# Autodesk Inventor assembly: компановка новая
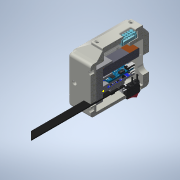
[picture p0: Inventor's stored thumbnail of the model, 180x180]
Saved by Autodesk Inventor 2021 (Build 250183000, 183)
## iProperties
Created: 2023-02-11
Part Number: компановка новая
Document SubType Name: Assembly
Designer: Tasya
Mass: 94.4631 g
Surface Area: 527.261 cm^2
Volume: 88.6889 cm^3
Density: 1.06511 g/cm^3
Author: Tasya
## Documents named in this file (6)
- C:\Users\Tasya\Desktop\теплица\3D модели\компановка новая.iam
- C:\Users\Tasya\Desktop\теплица\датчики почва воздух\корпус.ipt
- C:\Users\Tasya\Desktop\теплица\датчики почва воздух\DHT11.ipt
- C:\Users\Tasya\Desktop\теплица\датчики почва воздух\крышка корпус.ipt
- C:\Users\Tasya\Desktop\теплица\grabcad\Switch on off.ipt
- C:\Users\Tasya\Desktop\теплица\датчики почва воздух\Компоновка.iam
## Components (5 placed, 5 different names)
1. корпус:1 — Совмещение:1, Совмещение:2, Совмещение:3, Совмещение:4, Совмещение:8, Совмещение:9, Совмещение:11, Совмещение:12, Совмещение:13, Совмещение:14, Совмещение:15
2. DHT11:1 — Совмещение:1, Совмещение:2, Совмещение:3
3. крышка корпус:1 — Совмещение:4, Совмещение:8, Совмещение:9
4. Switch on off:1 — Совмещение:11, Совмещение:12, Совмещение:13
5. Компоновка:1 [sub-assembly] — Совмещение:10, Угол:1, Совмещение:14, Совмещение:15
## Relationships (13: Mate 12, Angle 1)
- Совмещение:1 [Mate] (1 mm): корпус:1 ↔ DHT11:1
- Совмещение:2 [Mate] (1 mm): корпус:1 ↔ DHT11:1
- Совмещение:3 [Mate] (0.5 mm): корпус:1 ↔ DHT11:1
- Совмещение:4 [Mate]: корпус:1 ↔ крышка корпус:1
- Совмещение:8 [Mate]: корпус:1 ↔ крышка корпус:1
- Совмещение:9 [Mate]: корпус:1 ↔ крышка корпус:1
- Совмещение:10 [Mate]: Компоновка:1
- Угол:1 [Angle] (180 deg): Компоновка:1
- Совмещение:11 [Mate]: корпус:1 ↔ Switch on off:1
- Совмещение:12 [Mate] (1.7 mm): корпус:1 ↔ Switch on off:1
- Совмещение:13 [Mate]: корпус:1 ↔ Switch on off:1
- Совмещение:14 [Mate]: корпус:1 ↔ Компоновка:1
- Совмещение:15 [Mate] (1 mm): корпус:1 ↔ Компоновка:1
